# Autodesk Inventor assembly: example
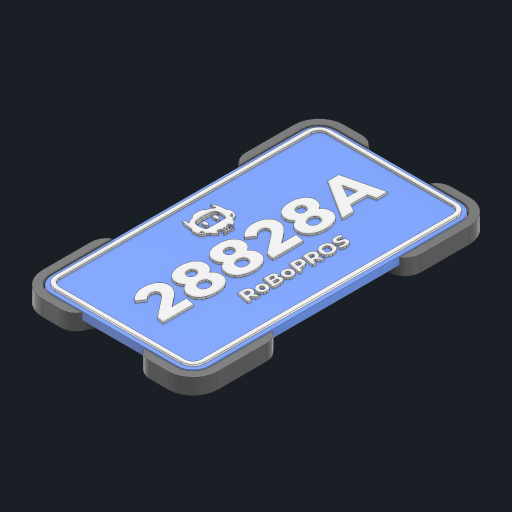
[picture p0: Inventor's stored thumbnail of the model, 512x512]
Saved by Autodesk Inventor 2024 (Build 280153000, 153)
## iProperties
Created: 2024-06-21
Part Number: example
Document SubType Name: Assembly
Designer: Averey Ku
Author: Averey Ku
## Documents named in this file (4)
- D:\vex_robotics_high_stakes\hardware\cad\magplate_final\example.iam
- D:\vex_robotics_high_stakes\hardware\cad\magplate_final\magplate_holder.ipt
- D:\vex_robotics_high_stakes\hardware\cad\magplate_final\magplate.iam
- magplate.iam
## Components (2 placed, 2 different names)
1. magplate_holder:1 — Insert:1, Mate:1
2. magplate:1 [sub-assembly] — Insert:1, Mate:1
## Relationships (2: Insert 1, Mate 1)
- Insert:1: magplate_holder:1 ↔ magplate:1
- Mate:1: magplate_holder:1 ↔ magplate:1
